# Autodesk Inventor assembly: Rover Main
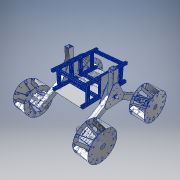
[picture p0: Inventor's stored thumbnail of the model, 180x180]
Saved by Autodesk Inventor 2019 (Build 230136000, 136)
## iProperties
Created: 2018-10-13
Part Number: Rover Main
Document SubType Name: Assembly
Designer: Adhik
Mass: 19209.4 g
Surface Area: 56367.3 cm^2
Volume: 7040.54 cm^3
Density: 2.72839 g/cm^3
Author: Adhik
## Documents named in this file (10)
- I:\CAD\Julie\Rover Main.iam
- I:\CAD\Julie\Baseplate.ipt
- I:\CAD\Julie\8020 20 inch lower.ipt
- I:\CAD\Julie\Lateral Plate.ipt
- I:\CAD\Julie\8020 12 inch.ipt
- I:\CAD\Julie\8020 20 inch upper.ipt
- I:\CAD\Julie\Main Joint.ipt
- I:\CAD\Julie\Main Axle.ipt
- I:\CAD\Julie\8020 6 inch.ipt
- I:\CAD\Julie\Drive Assembly.iam
## Components (24 placed, 9 different names)
1. Baseplate:1 — Flush:1, Flush:2, Mate:1, Mate:2, Flush:3, Flush:4, Flush:5, Flush:6, Mate:5, Mate:9
2. 8020 20 inch lower:1 — Mate:2, Flush:3, Flush:4, Mate:3, Mate:6, Mate:7, Mate:8, Mate:10, Flush:12, Mate:27, Mate:28, Mate:29, Mate:30
3. 8020 20 inch lower:2 — Flush:1, Flush:2, Mate:1, Mate:4, Flush:11, Mate:23, Mate:24, Mate:25, Mate:26
4. Lateral Plate:1 — Mate:3, Flush:5, Flush:7, Mate:12, Mate:15, Mate:19, Mate:20, Flush:26, Flush:27
5. Lateral Plate:2 — Mate:4, Flush:6, Flush:8, Mate:11, Mate:16, Mate:17, Mate:18, Flush:24, Flush:25
6. 8020 12 inch:1 — Mate:5, Mate:6, Mate:7
7. 8020 12 inch:2 — Mate:8, Mate:9, Mate:10
8. 8020 12 inch:3 — Mate:14, Flush:13, Flush:29, Mate:35, Mate:36
9. 8020 12 inch:4 — Mate:13, Flush:14, Flush:28, Mate:31, Mate:34
10. 8020 20 inch upper:1 — Mate:11, Flush:11, Mate:13, Mate:14, Flush:13, Flush:14, Flush:15, Flush:16, Flush:17, Flush:18, Flush:28, Mate:32
11. 8020 20 inch upper:2 — Mate:12, Flush:12, Flush:20, Flush:21, Flush:22, Flush:23, Mate:33, Flush:29
12. Main Joint:1 — Mate:16, Mate:17, Mate:18, Mate:40
13. Main Joint:2 — Mate:15, Mate:19, Mate:20, Mate:21, Mate:39
14. Main Axle:1 — Mate:21, Mate:22, Mate:37, Mate:38
15. 8020 6 inch:2 — Flush:16, Mate:24, Flush:24, Mate:32
16. 8020 6 inch:3 — Flush:23, Mate:30, Mate:34
17. 8020 6 inch:4 — Flush:21, Mate:28, Mate:35
18. 8020 6 inch:5 — Flush:15, Mate:25, Flush:25
19. 8020 6 inch:6 — Flush:22, Mate:29, Flush:27, Mate:33
20. 8020 6 inch:7 — Flush:17, Mate:26, Mate:36
21. 8020 6 inch:8 — Flush:20, Mate:27, Flush:26
22. 8020 6 inch:9 — Flush:18, Mate:23, Mate:31
23. Drive Assembly:1 [sub-assembly] — Mate:38, Mate:40
24. Drive Assembly:2 [sub-assembly] — Mate:37, Mate:39
## Relationships (66: Mate 40, Flush 26)
- Flush:1: Baseplate:1 ↔ 8020 20 inch lower:2
- Flush:2: Baseplate:1 ↔ 8020 20 inch lower:2
- Mate:1: Baseplate:1 ↔ 8020 20 inch lower:2
- Mate:2: Baseplate:1 ↔ 8020 20 inch lower:1
- Flush:3: Baseplate:1 ↔ 8020 20 inch lower:1
- Flush:4: Baseplate:1 ↔ 8020 20 inch lower:1
- Mate:3: 8020 20 inch lower:1 ↔ Lateral Plate:1
- Mate:4: 8020 20 inch lower:2 ↔ Lateral Plate:2
- Flush:5: Baseplate:1 ↔ Lateral Plate:1
- Flush:6: Baseplate:1 ↔ Lateral Plate:2
- Flush:7: Lateral Plate:1
- Flush:8: Lateral Plate:2
- Mate:5: Baseplate:1 ↔ 8020 12 inch:1
- Mate:6: 8020 20 inch lower:1 ↔ 8020 12 inch:1
- Mate:7: 8020 20 inch lower:1 ↔ 8020 12 inch:1
- Mate:8: 8020 20 inch lower:1 ↔ 8020 12 inch:2
- Mate:9: Baseplate:1 ↔ 8020 12 inch:2
- Mate:10: 8020 20 inch lower:1 ↔ 8020 12 inch:2
- Mate:11: Lateral Plate:2 ↔ 8020 20 inch upper:1
- Mate:12: Lateral Plate:1 ↔ 8020 20 inch upper:2
- Flush:11: 8020 20 inch lower:2 ↔ 8020 20 inch upper:1
- Flush:12: 8020 20 inch lower:1 ↔ 8020 20 inch upper:2
- Mate:13: 8020 12 inch:4 ↔ 8020 20 inch upper:1
- Mate:14: 8020 12 inch:3 ↔ 8020 20 inch upper:1
- Flush:13: 8020 12 inch:3 ↔ 8020 20 inch upper:1
- Flush:14: 8020 12 inch:4 ↔ 8020 20 inch upper:1
- Mate:15: Lateral Plate:1 ↔ Main Joint:2
- Mate:16: Lateral Plate:2 ↔ Main Joint:1
- Mate:17: Lateral Plate:2 ↔ Main Joint:1
- Mate:18: Lateral Plate:2 ↔ Main Joint:1
- Mate:19: Lateral Plate:1 ↔ Main Joint:2
- Mate:20: Lateral Plate:1 ↔ Main Joint:2
- Mate:21: Main Joint:2 ↔ Main Axle:1
- Mate:22: Main Axle:1
- Flush:15: 8020 20 inch upper:1 ↔ 8020 6 inch:5
- Flush:16: 8020 20 inch upper:1 ↔ 8020 6 inch:2
- Flush:17: 8020 20 inch upper:1 ↔ 8020 6 inch:7
- Flush:18: 8020 20 inch upper:1 ↔ 8020 6 inch:9
- Mate:23: 8020 20 inch lower:2 ↔ 8020 6 inch:9
- Mate:24: 8020 20 inch lower:2 ↔ 8020 6 inch:2
- Mate:25: 8020 20 inch lower:2 ↔ 8020 6 inch:5
- Mate:26: 8020 20 inch lower:2 ↔ 8020 6 inch:7
- Flush:20: 8020 20 inch upper:2 ↔ 8020 6 inch:8
- Flush:21: 8020 20 inch upper:2 ↔ 8020 6 inch:4
- Flush:22: 8020 20 inch upper:2 ↔ 8020 6 inch:6
- Flush:23: 8020 20 inch upper:2 ↔ 8020 6 inch:3
- Mate:27: 8020 20 inch lower:1 ↔ 8020 6 inch:8
- Mate:28: 8020 20 inch lower:1 ↔ 8020 6 inch:4
- Mate:29: 8020 20 inch lower:1 ↔ 8020 6 inch:6
- Mate:30: 8020 20 inch lower:1 ↔ 8020 6 inch:3
- Flush:24: Lateral Plate:2 ↔ 8020 6 inch:2
- Flush:25: Lateral Plate:2 ↔ 8020 6 inch:5
- Flush:26: Lateral Plate:1 ↔ 8020 6 inch:8
- Flush:27: Lateral Plate:1 ↔ 8020 6 inch:6
- Flush:28 (-25.4 mm): 8020 12 inch:4 ↔ 8020 20 inch upper:1
- Mate:31: 8020 12 inch:4 ↔ 8020 6 inch:9
- Mate:32: 8020 20 inch upper:1 ↔ 8020 6 inch:2
- Mate:33: 8020 20 inch upper:2 ↔ 8020 6 inch:6
- Mate:34: 8020 12 inch:4 ↔ 8020 6 inch:3
- Flush:29 (-25.4 mm): 8020 12 inch:3 ↔ 8020 20 inch upper:2
- Mate:35: 8020 12 inch:3 ↔ 8020 6 inch:4
- Mate:36: 8020 12 inch:3 ↔ 8020 6 inch:7
- Mate:37: Main Axle:1 ↔ Drive Assembly:2
- Mate:38: Main Axle:1 ↔ Drive Assembly:1
- Mate:39: Main Joint:2 ↔ Drive Assembly:2
- Mate:40: Main Joint:1 ↔ Drive Assembly:1
